# Autodesk Inventor assembly: 2 Omni AS, Circle
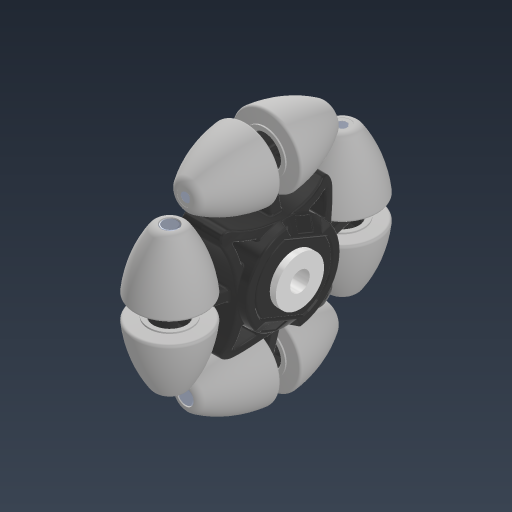
[picture p0: Inventor's stored thumbnail of the model, 512x512]
Saved by Autodesk Inventor 2024.3 (Build 283343000, 343)
## iProperties
Created: 2024-04-29
Part Number: 2 Omni AS, Circle
Document SubType Name: Assembly
Designer: chase
Author: chase
## Documents named in this file (3)
- C:\Users\chase\OneDrive\Desktop\VEX-CAD-Inventor\Motion\Wheels\Omni Wheel\2 Omni AS, Circle.iam
- C:\Users\chase\OneDrive\Desktop\VEX-CAD-Inventor\Motion\Wheels\Omni Wheel\2 Omni AS, No Insert.ipt
- C:\Users\chase\OneDrive\Desktop\VEX-CAD-Inventor\Motion\Insert Circle.ipt
## Components (3 placed, 2 different names)
1. 2 Omni AS, No Insert:1 — Insert:1, Angle:1, Insert:2, Angle:2
2. Insert Circle:2 — Insert:1, Angle:1
3. Insert Circle:1 — Insert:2, Angle:2
## Relationships (4: Insert 2, Angle 2)
- Insert:1: 2 Omni AS, No Insert:1 ↔ Insert Circle:2
- Angle:1 (0 deg): 2 Omni AS, No Insert:1 ↔ Insert Circle:2
- Insert:2: 2 Omni AS, No Insert:1 ↔ Insert Circle:1
- Angle:2 (0 deg): 2 Omni AS, No Insert:1 ↔ Insert Circle:1
